# Autodesk Inventor assembly: Shoulder Joint Assembly
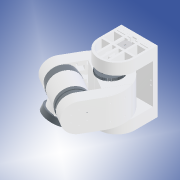
[picture p0: Inventor's stored thumbnail of the model, 180x180]
Saved by Autodesk Inventor 2017 SP1 (Build 210196100, 196)
## iProperties
Created: 2017-06-01
Part Number: Shoulder Joint Assembly
Document SubType Name: Assembly
Designer: Zach
Author: Zach
## Documents named in this file (16)
- C:\Users\Zach\Documents\GitHub\cr-laundry-robot\src\Body\Arm Assembly\Shoulder Joint Assembly\Shoulder Joint Assembly.iam
- C:\Users\Zach\Documents\GitHub\cr-laundry-robot\src\Body\Arm Assembly\Shoulder Joint Assembly\SJ002.ipt
- C:\Users\Zach\Documents\GitHub\cr-laundry-robot\src\Body\Arm Assembly\Shoulder Joint Assembly\SJ003.ipt
- C:\Users\Zach\Documents\GitHub\cr-laundry-robot\src\Body\Arm Assembly\Shoulder Joint Assembly\SJ001.ipt
- C:\Users\Zach\Documents\GitHub\cr-laundry-robot\lib\Stepper Motor - NEMA 17\NEMA17.ipt
- C:\Users\Zach\Documents\GitHub\cr-laundry-robot\src\Body\Arm Assembly\Shoulder Joint Assembly\SJ004.ipt
- C:\Users\Zach\Documents\GitHub\cr-laundry-robot\src\Body\Arm Assembly\Shoulder Joint Assembly\SJ005.ipt
- C:\Users\Zach\Documents\GitHub\cr-laundry-robot\src\Body\Arm Assembly\Shoulder Joint Assembly\SJ006.ipt
- C:\Users\Zach\Documents\GitHub\cr-laundry-robot\lib\U51105\U51105.ipt
- C:\Users\Zach\Documents\GitHub\cr-laundry-robot\lib\QS12MM250\QS12MM250.ipt
- C:\Users\Zach\Documents\GitHub\cr-laundry-robot\lib\6201RS\6201RS.ipt
- C:\Users\Zach\Documents\GitHub\cr-laundry-robot\src\Body\Arm Assembly\Shoulder Joint Assembly\SJ007.ipt
- C:\Users\Zach\Documents\GitHub\cr-laundry-robot\src\Body\Arm Assembly\Shoulder Joint Assembly\SJ008.ipt
- C:\Users\Zach\Documents\GitHub\cr-laundry-robot\src\Body\Arm Assembly\Shoulder Joint Assembly\Shoulder Joint Assembly\Design Accelerator\Spur Gears1.iam
- C:\Users\Zach\Documents\GitHub\cr-laundry-robot\src\Body\Arm Assembly\Shoulder Joint Assembly\SJ009.ipt
- C:\Users\Zach\Documents\GitHub\cr-laundry-robot\lib\46_1 Harmonic Drive Gearbox\46_1 Harmonic Drive Assembly.iam
## Components (27 placed, 15 different names)
1. SJ001:1 — Mate:47, Mate:48, Mate:49, Mate:152, Mate:157, Mate:158
2. SJ001:2 — Mate:159, Mate:160, Mate:161, Mate:162
3. SJ002:1 — Mate:1, Mate:4, Mate:8, Mate:9, Mate:153, Mate:156
4. SJ002:2 — Mate:18, Mate:19, Mate:20, Mate:154, Mate:155
5. SJ003:1 — Mate:1, Mate:4, Mate:8, Mate:9, Mate:18, Mate:19, Mate:20, Mate:145, Mate:147, Mate:148, Mate:149, Mate:150, Mate:151
6. SJ004:1 — Mate:130, Mate:140, Mate:141, Mate:160, Mate:162, Mate:163
7. SJ004:2 — Mate:47, Mate:48, Mate:49, Mate:54, Mate:55, Mate:56, Mate:142, Mate:143
8. SJ005:1 — Mate:54, Mate:55, Mate:56, Mate:60, Mate:67, Mate:69, Mate:70, Mate:80, Flush:1
9. SJ005:2 — Mate:68, Mate:82, Mate:84, Mate:130, Mate:135, Mate:136, Flush:1, Mate:163
10. SJ006:2 — Mate:67, Mate:68, Mate:69, Mate:70, Mate:78, Mate:79, Mate:83
11. NEMA17:3 — Mate:148, Mate:149, Mate:150
12. U51105:1 — Mate:131, Mate:139
13. U51105:2 — Mate:78, Mate:79
14. QS12MM250:1 — Mate:80, Mate:105, Mate:117, Mate:119, Mate:120, Mate:132, Mate:134
15. 6201RS:1 — Mate:82, Mate:138
16. 6201RS:2 — Mate:83, Mate:84
17. SJ007:1 — Mate:121, Mate:122, Mate:123, Mate:133
18. SJ008:1 — Mate:119, Mate:125, Mate:126, Mate:127, Mate:132
19. SJ008:2 — Mate:97, Mate:98, Mate:99, Mate:105, Mate:112, Mate:117, Mate:120, Mate:121, Mate:122, Mate:123, Mate:124, Mate:131
20. NEMA17:4 — Mate:97, Mate:98, Mate:99, Mate:137
21. SJ007:2 — Mate:125, Mate:126, Mate:127, Mate:133
22. Spur Gears:1 [sub-assembly] — Mate:134, Mate:135, Mate:136, Mate:137, Mate:138, Mate:139
23. SJ009:1 — Mate:140, Mate:141
24. SJ009:2 — Mate:142, Mate:143
25. 46_1 Harmonic Drive Assembly:1 [sub-assembly] — Mate:145, Mate:147, Mate:151
26. 46_1 Harmonic Drive Assembly:2 [sub-assembly] — Mate:152, Mate:153, Mate:156, Mate:157, Mate:158
27. 46_1 Harmonic Drive Assembly:3 [sub-assembly] — Mate:154, Mate:155, Mate:159, Mate:161
## Relationships (72: Mate 71, Flush 1)
- Mate:1: SJ002:1 ↔ SJ003:1
- Mate:4: SJ002:1 ↔ SJ003:1
- Mate:8: SJ002:1 ↔ SJ003:1
- Mate:9: SJ002:1 ↔ SJ003:1
- Mate:18: SJ002:2 ↔ SJ003:1
- Mate:19: SJ002:2 ↔ SJ003:1
- Mate:20: SJ002:2 ↔ SJ003:1
- Mate:47: SJ001:1 ↔ SJ004:2
- Mate:48: SJ001:1 ↔ SJ004:2
- Mate:49: SJ001:1 ↔ SJ004:2
- Mate:54: SJ004:2 ↔ SJ005:1
- Mate:55: SJ004:2 ↔ SJ005:1
- Mate:56: SJ004:2 ↔ SJ005:1
- Mate:60: SJ005:1
- Mate:67: SJ005:1 ↔ SJ006:2
- Mate:68: SJ005:2 ↔ SJ006:2
- Mate:69: SJ005:1 ↔ SJ006:2
- Mate:70: SJ005:1 ↔ SJ006:2
- Mate:78: SJ006:2 ↔ U51105:2
- Mate:79: SJ006:2 ↔ U51105:2
- Mate:80: SJ005:1 ↔ QS12MM250:1
- Mate:82: SJ005:2 ↔ 6201RS:1
- Mate:83: SJ006:2 ↔ 6201RS:2
- Mate:84: SJ005:2 ↔ 6201RS:2
- Mate:97: SJ008:2 ↔ NEMA17:4
- Mate:98: SJ008:2 ↔ NEMA17:4
- Mate:99: SJ008:2 ↔ NEMA17:4
- Mate:105: QS12MM250:1 ↔ SJ008:2
- Mate:112: SJ008:2
- Mate:117: QS12MM250:1 ↔ SJ008:2
- Mate:119: QS12MM250:1 ↔ SJ008:1
- Mate:120: QS12MM250:1 ↔ SJ008:2
- Mate:121: SJ007:1 ↔ SJ008:2
- Mate:122: SJ007:1 ↔ SJ008:2
- Mate:123: SJ007:1 ↔ SJ008:2
- Mate:124: SJ008:2
- Mate:125: SJ008:1 ↔ SJ007:2
- Mate:126: SJ008:1 ↔ SJ007:2
- Mate:127: SJ008:1 ↔ SJ007:2
- Mate:130: SJ004:1 ↔ SJ005:2
- Mate:131: U51105:1 ↔ SJ008:2
- Mate:132: QS12MM250:1 ↔ SJ008:1
- Mate:133: SJ007:1 ↔ SJ007:2
- Mate:134: QS12MM250:1 ↔ Spur Gears:1
- Mate:135: SJ005:2 ↔ Spur Gears:1
- Mate:136: SJ005:2 ↔ Spur Gears:1
- Mate:137: NEMA17:4 ↔ Spur Gears:1
- Mate:138: 6201RS:1 ↔ Spur Gears:1
- Mate:139: U51105:1 ↔ Spur Gears:1
- Mate:140: SJ004:1 ↔ SJ009:1
- Mate:141: SJ004:1 ↔ SJ009:1
- Mate:142: SJ004:2 ↔ SJ009:2
- Mate:143: SJ004:2 ↔ SJ009:2
- Mate:145: SJ003:1 ↔ 46_1 Harmonic Drive Assembly:1
- Mate:147: SJ003:1 ↔ 46_1 Harmonic Drive Assembly:1
- Mate:148: SJ003:1 ↔ NEMA17:3
- Mate:149: SJ003:1 ↔ NEMA17:3
- Mate:150: SJ003:1 ↔ NEMA17:3
- Mate:151: SJ003:1 ↔ 46_1 Harmonic Drive Assembly:1
- Mate:152: SJ001:1 ↔ 46_1 Harmonic Drive Assembly:2
- Mate:153: SJ002:1 ↔ 46_1 Harmonic Drive Assembly:2
- Mate:154: SJ002:2 ↔ 46_1 Harmonic Drive Assembly:3
- Mate:155: SJ002:2 ↔ 46_1 Harmonic Drive Assembly:3
- Mate:156: SJ002:1 ↔ 46_1 Harmonic Drive Assembly:2
- Mate:157: SJ001:1 ↔ 46_1 Harmonic Drive Assembly:2
- Mate:158: SJ001:1 ↔ 46_1 Harmonic Drive Assembly:2
- Mate:159: SJ001:2 ↔ 46_1 Harmonic Drive Assembly:3
- Mate:160: SJ001:2 ↔ SJ004:1
- Mate:161: SJ001:2 ↔ 46_1 Harmonic Drive Assembly:3
- Mate:162: SJ001:2 ↔ SJ004:1
- Flush:1: SJ005:1 ↔ SJ005:2
- Mate:163: SJ004:1 ↔ SJ005:2
